# Autodesk Inventor assembly: Tilting head
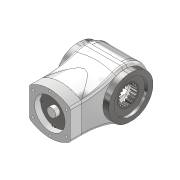
[picture p0: Inventor's stored thumbnail of the model, 180x180]
Saved by Autodesk Inventor 2020.3 (Build 243373010, 373A)
## iProperties
Created: 2021-05-11
Part Number: Tilting head
Document SubType Name: Assembly
Designer: marti
Author: marti
## Documents named in this file (9)
- C:\Users\marti\Documents\Inventor\RobotManipulateArm\17.4.2021 - Complete new IDEA\Tilting head.iam
- C:\Users\marti\Documents\Inventor\RobotManipulateArm\17.4.2021 - Complete new IDEA\Tilting unit of head.ipt
- C:\Users\marti\Documents\Inventor\RobotManipulateArm\17.4.2021 - Complete new IDEA\Servo\Servo 250 W.iam
- C:\Users\marti\Documents\Inventor\RobotManipulateArm\17.4.2021 - Complete new IDEA\Planetery gearbox.iam
- C:\Users\marti\Documents\Inventor\RobotManipulateArm\17.4.2021 - Complete new IDEA\Tilting head - extended part.ipt
- C:\Users\marti\Documents\Inventor\RobotManipulateArm\17.4.2021 - Complete new IDEA\Tilting head - cover side part.ipt
- C:\Users\marti\Documents\Inventor\RobotManipulateArm\17.4.2021 - Complete new IDEA\Head gear shaft Inner for shaft n.2.iam
- C:\Users\marti\Documents\Inventor\RobotManipulateArm\17.4.2021 - Complete new IDEA\Back cover of tilting head.ipt
- C:\Users\marti\Documents\Inventor\RobotManipulateArm\17.4.2021 - Complete new IDEA\Midlle inner console for tilting head.ipt
## Components (11 placed, 8 different names)
1. Tilting unit of head:1 — Angle:1, Mate:9, Mate:10, Mate:11, Mate:13, Mate:14, Angle:2, Mate:15, Mate:16, Mate:18, Mate:19, Mate:22, Mate:23, Mate:24, Mate:25, Mate:26, Mate:27, Mate:28, Mate:29, Mate:30, Flush:4, Mate:31, Mate:33, Mate:35
2. Servo 250 W:1 [sub-assembly] — Mate:2, Angle:1, Mate:5, Flush:4, Mate:32, Mate:34
3. Planetery gearbox:1 [sub-assembly] — Mate:34, Mate:35
4. Tilting head - extended part:1 — Mate:28, Mate:29, Mate:30
5. Tilting head - cover side part:1 — Mate:12, Mate:13, Mate:14, Angle:2, Mate:15, Mate:17, Mate:20, Flush:2
6. Tilting head - cover side part:2 — Mate:17, Mate:18, Mate:19, Mate:21, Flush:3
7. Head gear shaft Inner for shaft n.2:1 [sub-assembly] — Mate:21, Flush:3
8. Head gear shaft Inner for shaft n.2:2 [sub-assembly] — Mate:20, Flush:2
9. Back cover of tilting head:1 — Mate:22, Mate:23, Mate:24
10. Midlle inner console for tilting head:2 — Mate:31, Mate:32, Mate:33
11. Midlle inner console for tilting head:3 — Mate:25, Mate:26
## Relationships (34: Mate 29, Flush 3, Angle 2)
- Mate:2: Servo 250 W:1
- Angle:1 (0 deg): Tilting unit of head:1 ↔ Servo 250 W:1
- Mate:5: Servo 250 W:1
- Mate:9: Tilting unit of head:1
- Mate:10: Tilting unit of head:1
- Mate:11: Tilting unit of head:1
- Mate:12: Tilting head - cover side part:1
- Mate:13: Tilting unit of head:1 ↔ Tilting head - cover side part:1
- Mate:14: Tilting unit of head:1 ↔ Tilting head - cover side part:1
- Angle:2 (0 deg): Tilting unit of head:1 ↔ Tilting head - cover side part:1
- Mate:15: Tilting unit of head:1 ↔ Tilting head - cover side part:1
- Mate:16: Tilting unit of head:1
- Mate:17: Tilting head - cover side part:1 ↔ Tilting head - cover side part:2
- Mate:18: Tilting unit of head:1 ↔ Tilting head - cover side part:2
- Mate:19: Tilting unit of head:1 ↔ Tilting head - cover side part:2
- Mate:20: Tilting head - cover side part:1 ↔ Head gear shaft Inner for shaft n.2:2
- Flush:2: Tilting head - cover side part:1 ↔ Head gear shaft Inner for shaft n.2:2
- Mate:21: Tilting head - cover side part:2 ↔ Head gear shaft Inner for shaft n.2:1
- Flush:3: Tilting head - cover side part:2 ↔ Head gear shaft Inner for shaft n.2:1
- Mate:22: Tilting unit of head:1 ↔ Back cover of tilting head:1
- Mate:23: Tilting unit of head:1 ↔ Back cover of tilting head:1
- Mate:24: Tilting unit of head:1 ↔ Back cover of tilting head:1
- Mate:25: Tilting unit of head:1 ↔ Midlle inner console for tilting head:3
- Mate:26: Tilting unit of head:1 ↔ Midlle inner console for tilting head:3
- Mate:27: Tilting unit of head:1
- Mate:28: Tilting unit of head:1 ↔ Tilting head - extended part:1
- Mate:29: Tilting unit of head:1 ↔ Tilting head - extended part:1
- Mate:30: Tilting unit of head:1 ↔ Tilting head - extended part:1
- Flush:4: Tilting unit of head:1 ↔ Servo 250 W:1
- Mate:31: Tilting unit of head:1 ↔ Midlle inner console for tilting head:2
- Mate:32: Servo 250 W:1 ↔ Midlle inner console for tilting head:2
- Mate:33: Tilting unit of head:1 ↔ Midlle inner console for tilting head:2
- Mate:34: Servo 250 W:1 ↔ Planetery gearbox:1
- Mate:35: Tilting unit of head:1 ↔ Planetery gearbox:1
